# Autodesk Inventor assembly: hooks and faceplate
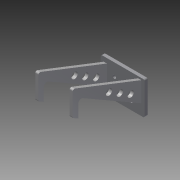
[picture p0: Inventor's stored thumbnail of the model, 180x180]
Saved by Autodesk Inventor 2013 (Build 170138000, 138)
## iProperties
Created: 2013-02-10
Part Number: hooks and faceplate
Document SubType Name: Weldment
Designer: Arpan
Weld Material: Welded Aluminum-6061
Author: Arpan
## Documents named in this file (3)
- C:\Users\Arpan\Documents\GitHub\frc2013CAD\hooks and faceplate.iam
- C:\Users\Arpan\Documents\GitHub\frc2013CAD\Cimber actual\hook faceplate.ipt
- C:\Users\Arpan\Documents\GitHub\frc2013CAD\Cimber actual\hook.ipt
## Components (3 placed, 2 different names)
1. hook faceplate:1 — Mate:1, Mate:2, Mate:3, Mate:4
2. hook:1 — Mate:1, Mate:2
3. hook:2 — Mate:3, Mate:4
## Relationships (4: Mate 4)
- Mate:1: hook faceplate:1 ↔ hook:1
- Mate:2: hook faceplate:1 ↔ hook:1
- Mate:3: hook faceplate:1 ↔ hook:2
- Mate:4: hook faceplate:1 ↔ hook:2
